# Autodesk Inventor assembly: Z-axis Left Plate
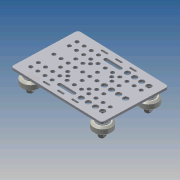
[picture p0: Inventor's stored thumbnail of the model, 180x180]
Saved by Autodesk Inventor 2015 (Build 190159000, 159)
## iProperties
Created: 2015-10-03
Part Number: Z-axis Left Plate
Document SubType Name: Assembly
Designer: Solomon
Author: Solomon
## Documents named in this file (3)
- C:\Users\Solomon\Documents\Inventor\Omni 1\X-carriage.iam
- C:\Users\Solomon\Documents\Inventor\Omni 1\V Slot Part Files\V Slot Plates\Large Build Plate.ipt
- C:\Users\Solomon\Documents\Inventor\Omni 1\V Slot Part Files\assembledwheel.iam
## Components (5 placed, 2 different names)
1. Large Build Plate:2 — Mate:1, Mate:2, Mate:3, Mate:4, Angle:3, Angle:4, Angle:5, Angle:6
2. assembledwheel:1 [sub-assembly] — Mate:1, Angle:5
3. assembledwheel:2 [sub-assembly] — Mate:2, Angle:6
4. assembledwheel:3 [sub-assembly] — Mate:3, Angle:3
5. assembledwheel:4 [sub-assembly] — Mate:4, Angle:4
## Relationships (8: Mate 4, Angle 4)
- Mate:1: Large Build Plate:2 ↔ assembledwheel:1
- Mate:2: Large Build Plate:2 ↔ assembledwheel:2
- Mate:3: Large Build Plate:2 ↔ assembledwheel:3
- Mate:4: Large Build Plate:2 ↔ assembledwheel:4
- Angle:3 (0 deg): Large Build Plate:2 ↔ assembledwheel:3
- Angle:4 (0 deg): Large Build Plate:2 ↔ assembledwheel:4
- Angle:5 (0 deg): Large Build Plate:2 ↔ assembledwheel:1
- Angle:6 (0 deg): Large Build Plate:2 ↔ assembledwheel:2
